# Autodesk Inventor assembly: Assembly1
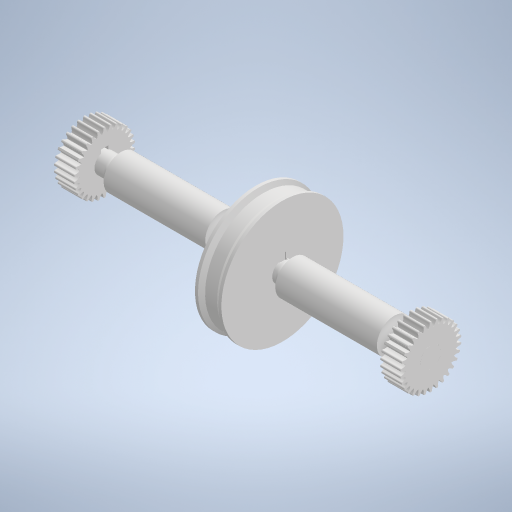
[picture p0: Inventor's stored thumbnail of the model, 512x512]
Saved by Autodesk Inventor 2024 (Build 280153000, 153)
## iProperties
Created: 2024-03-20
Part Number: Assembly1
Document SubType Name: Assembly
Designer: di18e
Author: di18e
## Documents named in this file (5)
- C:\Users\di18e\Desktop\Assembly1.iam
- C:\Users\di18e\Downloads\ENGRANE.ipt
- C:\Users\di18e\Downloads\POLEA.ipt
- C:\Users\di18e\Downloads\EJE_CUÑEROS.ipt
- C:\Users\di18e\Downloads\CUÑA.ipt
## Components (8 placed, 4 different names)
1. POLEA:1 — Mate:1, Flush:1, Mate:4, Mate:5, Flush:4
2. EJE_CUÑEROS:1 — Mate:1, Flush:1, Mate:3, Flush:3, Flush:5, Flush:6, Mate:7
3. ENGRANE:1 — Mate:3, Flush:3, Mate:6, Flush:5
4. CUÑA:2 — Mate:4
5. CUÑA:3 — Mate:5, Flush:4
6. CUÑA:4 — Mate:6, Flush:6
7. EJE_CUÑEROS:2 — Mate:7, Mate:8, Flush:7
8. ENGRANE:2 — Mate:8, Flush:7
## Relationships (13: Mate 7, Flush 6)
- Mate:1: POLEA:1 ↔ EJE_CUÑEROS:1
- Flush:1: POLEA:1 ↔ EJE_CUÑEROS:1
- Mate:3: EJE_CUÑEROS:1 ↔ ENGRANE:1
- Flush:3: EJE_CUÑEROS:1 ↔ ENGRANE:1
- Mate:4: POLEA:1 ↔ CUÑA:2
- Mate:5: POLEA:1 ↔ CUÑA:3
- Flush:4: POLEA:1 ↔ CUÑA:3
- Mate:6: ENGRANE:1 ↔ CUÑA:4
- Flush:5: EJE_CUÑEROS:1 ↔ ENGRANE:1
- Flush:6: EJE_CUÑEROS:1 ↔ CUÑA:4
- Mate:7: EJE_CUÑEROS:1 ↔ EJE_CUÑEROS:2
- Mate:8: EJE_CUÑEROS:2 ↔ ENGRANE:2
- Flush:7: EJE_CUÑEROS:2 ↔ ENGRANE:2
